# Autodesk Inventor assembly: RPLIDAR_A1
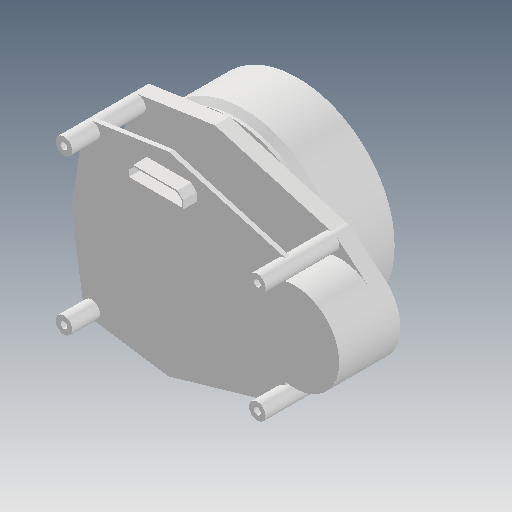
[picture p0: Inventor's stored thumbnail of the model, 512x512]
Saved by Autodesk Inventor 2020 (Build 240168000, 168)
## iProperties
Created: 2020-08-31
Part Number: RPLIDAR_A1
Document SubType Name: Assembly
Designer: 이호석
Mass: 180 g
Surface Area: 400.209 cm^2
Volume: 144.547 cm^3
Density: 1.24527 g/cm^3
Author: 이호석
## Documents named in this file (4)
- C:\Inventor\Embedded_contest\LIDAR\RPLIDAR_A1.iam
- C:\Inventor\Embedded_contest\LIDAR\base.ipt
- C:\Inventor\Embedded_contest\LIDAR\sensor.ipt
- C:\Inventor\Embedded_contest\LIDAR\wheel.ipt
## Components (3 placed, 3 different names)
1. base:1 — 삽입:1, 삽입:2
2. sensor:1 — 삽입:1
3. wheel:1 — 삽입:2
## Relationships (2: Insert 2)
- 삽입:1 [Insert]: base:1 ↔ sensor:1
- 삽입:2 [Insert]: base:1 ↔ wheel:1
